# Autodesk Inventor assembly: UNLHEP-14-01-A-010_GlueResOnChuck
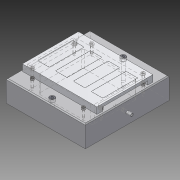
[picture p0: Inventor's stored thumbnail of the model, 180x180]
Saved by Autodesk Inventor 2013 (Build 170138000, 138)
## iProperties
Created: 2014-01-23
Part Number: UNLHEP-14-01-A-010_GlueResOnChuck
Document SubType Name: Assembly
Designer: Frank Meier
Author: Frank Meier
## Documents named in this file (6)
- C:\Users\Frank Meier\Documents\Inventor\Delvotec-Saugplatte\UNLHEP-14-01-A-010_GlueResOnChuck.iam
- C:\Users\Frank Meier\Documents\Inventor\Delvotec-Saugplatte\UNLHEP-14-01-P-004_ChuckForGantry.ipt
- C:\Users\Frank Meier\Documents\Inventor\Delvotec-Saugplatte\UNLHEP-14-01-P-017_GlueReservoit.ipt
- C:\Users\Frank Meier\Documents\Inventor\Delvotec-Saugplatte\UNLHEP-14-01-P-003_Tube4mmID20mm.ipt
- C:\Users\Frank Meier\Documents\Inventor\Content Center Files\R2013\de-DE\ANSI B18.3(05)\ANSI B18.3 - 1_4-20 UNC - 2(31).ipt
- C:\Users\Frank Meier\Documents\Inventor\Content Center Files\R2013\de-DE\ISO 4762(2)\ISO 4762 - M4 x 16ISO.ipt
## Components (13 placed, 5 different names)
1. UNLHEP-14-01-P-004_ChuckForGantry:1 — Passend:1, Passend:2, Passend:3, Passend:4, Passend:5, Passend:6, Passend:7, Einfügen:1, Einfügen:2, Einfügen:3, Einfügen:4, Einfügen:5, Einfügen:6, Einfügen:7, Einfügen:8
2. UNLHEP-14-01-P-017_GlueReservoit:1 — Passend:1
3. UNLHEP-14-01-P-003_Tube4mmID20mm:1 — Passend:2, Passend:3
4. Innensechskantschraube - Zoll 1/4 - 20 UNC - 2:1 — Passend:4, Passend:5
5. Innensechskantschraube - Zoll 1/4 - 20 UNC - 2:2 — Passend:6, Passend:7
6. ISO 4762 M4 x 16:1 — Einfügen:1
7. ISO 4762 M4 x 16:2 — Einfügen:2
8. ISO 4762 M4 x 16:3 — Einfügen:3
9. ISO 4762 M4 x 16:4 — Einfügen:4
10. ISO 4762 M4 x 16:5 — Einfügen:5
11. ISO 4762 M4 x 16:6 — Einfügen:6
12. ISO 4762 M4 x 16:7 — Einfügen:7
13. ISO 4762 M4 x 16:8 — Einfügen:8
## Relationships (15: Insert 8, Mate 7)
- Passend:1 [Mate]: UNLHEP-14-01-P-004_ChuckForGantry:1 ↔ UNLHEP-14-01-P-017_GlueReservoit:1
- Passend:2 [Mate]: UNLHEP-14-01-P-004_ChuckForGantry:1 ↔ UNLHEP-14-01-P-003_Tube4mmID20mm:1
- Passend:3 [Mate]: UNLHEP-14-01-P-004_ChuckForGantry:1 ↔ UNLHEP-14-01-P-003_Tube4mmID20mm:1
- Passend:5 [Mate]: UNLHEP-14-01-P-004_ChuckForGantry:1 ↔ Innensechskantschraube - Zoll 1/4 - 20 UNC - 2:1
- Passend:7 [Mate]: UNLHEP-14-01-P-004_ChuckForGantry:1 ↔ Innensechskantschraube - Zoll 1/4 - 20 UNC - 2:2
- Passend:4 [Mate]: UNLHEP-14-01-P-004_ChuckForGantry:1 ↔ Innensechskantschraube - Zoll 1/4 - 20 UNC - 2:1
- Passend:6 [Mate]: UNLHEP-14-01-P-004_ChuckForGantry:1 ↔ Innensechskantschraube - Zoll 1/4 - 20 UNC - 2:2
- Einfügen:1 [Insert]: UNLHEP-14-01-P-004_ChuckForGantry:1 ↔ ISO 4762 M4 x 16:1
- Einfügen:2 [Insert]: UNLHEP-14-01-P-004_ChuckForGantry:1 ↔ ISO 4762 M4 x 16:2
- Einfügen:3 [Insert]: UNLHEP-14-01-P-004_ChuckForGantry:1 ↔ ISO 4762 M4 x 16:3
- Einfügen:4 [Insert]: UNLHEP-14-01-P-004_ChuckForGantry:1 ↔ ISO 4762 M4 x 16:4
- Einfügen:5 [Insert]: UNLHEP-14-01-P-004_ChuckForGantry:1 ↔ ISO 4762 M4 x 16:5
- Einfügen:6 [Insert]: UNLHEP-14-01-P-004_ChuckForGantry:1 ↔ ISO 4762 M4 x 16:6
- Einfügen:7 [Insert]: UNLHEP-14-01-P-004_ChuckForGantry:1 ↔ ISO 4762 M4 x 16:7
- Einfügen:8 [Insert]: UNLHEP-14-01-P-004_ChuckForGantry:1 ↔ ISO 4762 M4 x 16:8
